# Autodesk Inventor assembly: StepperWithMount
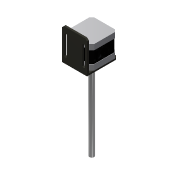
[picture p0: Inventor's stored thumbnail of the model, 180x180]
Saved by Autodesk Inventor 2014 (Build 180170000, 170)
## iProperties
Created: 2014-08-10
Part Number: StepperWithMount
Document SubType Name: Assembly
Designer: Peele
Author: Peele
## Documents named in this file (3)
- E:\Copy\DLP\PandaPrint\SubAssem\StepperWithMount.iam
- E:\Copy\DLP\PandaPrint\StockParts\StepperMount.ipt
- E:\Copy\DLP\PandaPrint\StockParts\StepperDrive.ipt
## Components (2 placed, 2 different names)
1. StepperMount:1 — Mate:1, Mate:2, Mate:3
2. StepperDrive:1 — Mate:1, Mate:2, Mate:3
## Relationships (3: Mate 3)
- Mate:1: StepperMount:1 ↔ StepperDrive:1
- Mate:2: StepperMount:1 ↔ StepperDrive:1
- Mate:3: StepperMount:1 ↔ StepperDrive:1
